# Autodesk Inventor assembly: ベアリング
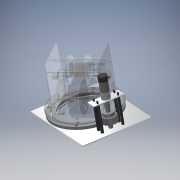
[picture p0: Inventor's stored thumbnail of the model, 180x180]
Saved by Autodesk Inventor 2019 (Build 230136000, 136)
## iProperties
Created: 2020-09-30
Part Number: ベアリング
Material: 一般
Document SubType Name: Assembly
Designer: Toshihito
Author: Toshihito
## Documents named in this file (12)
- C:\Users\zhept\OneDrive\大学\rrst\足回り2020\足回り試作2020_v1\足回り試作.iam
- 足回り2020v1.iam
- C:\Users\zhept\OneDrive\大学\rrst\足回り2020\足回り試作2020_v1\ベアリング 外側.ipt
- C:\Users\zhept\OneDrive\大学\rrst\足回り2020\足回り試作2020_v1\ベアリング 内側.ipt
- C:\Users\zhept\OneDrive\大学\rrst\足回り2020\足回り試作2020_v1\ベアリング板.ipt
- C:\Users\zhept\OneDrive\大学\rrst\足回り2020\足回り試作2020_v1\上層部.iam
- C:\Users\zhept\OneDrive\大学\rrst\足回り2020\足回り試作2020_v1\25d-metal-gearmotor-20.4-encoder.ipt
- C:\Users\zhept\OneDrive\大学\rrst\足回り2020\足回り試作2020_v1\SS2-20J12_On.ipt
- C:\Users\zhept\OneDrive\大学\rrst\足回り2020\足回り試作2020_v1\円柱12mm.ipt
- C:\Users\zhept\OneDrive\大学\rrst\足回り2020\足回り試作2020_v1\4mm-8mmカップリング.ipt
- C:\Users\zhept\OneDrive\大学\rrst\足回り2020\足回り試作2020_v1\板 中心Φ7.ipt
- C:\Users\zhept\OneDrive\大学\rrst\足回り2020\足回り試作2020_v1\六角支柱_回転モータ.ipt
## Components (13 placed, 10 different names)
1. ベアリング 外側:1 — フラッシュ:1, メイト:2, 挿入:1, 挿入:2
2. ベアリング 内側:1 — フラッシュ:1, メイト:1, フラッシュ:2, 挿入:3, 挿入:4
3. ベアリング板:1 — 挿入:1, 挿入:2, 挿入:9, 挿入:14, 挿入:15, 挿入:16, 挿入:17
4. 上層部:1 [sub-assembly] — 挿入:3, 挿入:4, フラッシュ:3, 角度:1
5. 25d-metal-gearmotor-20.4-encoder:1 — 挿入:6, 挿入:7, 挿入:8
6. SS2-20J12_On:1 — フラッシュ:3, メイト:4, 円柱状:1
7. 円柱12mm:1 — リジッド:1, 円柱状:1, 挿入:9
8. 4mm-8mmカップリング:1 — リジッド:1, 挿入:6
9. 板 中心Φ7:1 — 挿入:7, 挿入:8, 挿入:10, 挿入:11, 挿入:12, 挿入:13
10. 六角支柱_回転モータ:1 — 挿入:10, 挿入:16
11. 六角支柱_回転モータ:2 — 挿入:11, 挿入:15
12. 六角支柱_回転モータ:3 — 挿入:12, 挿入:14
13. 六角支柱_回転モータ:4 — 挿入:13, 挿入:17
## Relationships (26: Insert 16, Mate 4, Flush 3, Angle 1, WeldJoint 1, CylindricalJoint 1)
- フラッシュ:1 [Flush]: ベアリング 外側:1 ↔ ベアリング 内側:1
- メイト:1 [Mate]: ベアリング 内側:1
- メイト:2 [Mate]: ベアリング 外側:1
- フラッシュ:2 [Flush]: ベアリング 内側:1
- 挿入:1 [Insert] (2 mm): ベアリング 外側:1 ↔ ベアリング板:1
- 挿入:2 [Insert] (2 mm): ベアリング 外側:1 ↔ ベアリング板:1
- 挿入:3 [Insert] (5 mm): ベアリング 内側:1 ↔ 上層部:1
- 挿入:4 [Insert] (5 mm): ベアリング 内側:1 ↔ 上層部:1
- フラッシュ:3 [Flush]: 上層部:1 ↔ SS2-20J12_On:1
- 角度:1 [Angle] (0 deg): 上層部:1
- メイト:4 [Mate]: SS2-20J12_On:1
- リジッド:1 [WeldJoint]: 円柱12mm:1 ↔ 4mm-8mmカップリング:1
- 円柱状:1 [CylindricalJoint]: SS2-20J12_On:1 ↔ 円柱12mm:1
- メイト:5 [Mate] (120 mm)
- 挿入:6 [Insert] (1 mm): 25d-metal-gearmotor-20.4-encoder:1 ↔ 4mm-8mmカップリング:1
- 挿入:7 [Insert]: 25d-metal-gearmotor-20.4-encoder:1 ↔ 板 中心Φ7:1
- 挿入:8 [Insert]: 25d-metal-gearmotor-20.4-encoder:1 ↔ 板 中心Φ7:1
- 挿入:9 [Insert] (-2.5 mm): ベアリング板:1 ↔ 円柱12mm:1
- 挿入:10 [Insert]: 板 中心Φ7:1 ↔ 六角支柱_回転モータ:1
- 挿入:11 [Insert]: 板 中心Φ7:1 ↔ 六角支柱_回転モータ:2
- 挿入:12 [Insert]: 板 中心Φ7:1 ↔ 六角支柱_回転モータ:3
- 挿入:13 [Insert]: 板 中心Φ7:1 ↔ 六角支柱_回転モータ:4
- 挿入:14 [Insert]: ベアリング板:1 ↔ 六角支柱_回転モータ:3
- 挿入:15 [Insert]: ベアリング板:1 ↔ 六角支柱_回転モータ:2
- 挿入:16 [Insert]: ベアリング板:1 ↔ 六角支柱_回転モータ:1
- 挿入:17 [Insert]: ベアリング板:1 ↔ 六角支柱_回転モータ:4
